# Autodesk Inventor assembly: Assembled box
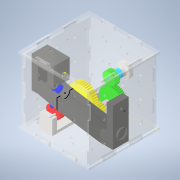
[picture p0: Inventor's stored thumbnail of the model, 180x180]
Saved by Autodesk Inventor 2021 (Build 250183000, 183)
## iProperties
Created: 2020-02-27
Part Number: Assembled box
Document SubType Name: Assembly
Designer: jstr255
Author: jstr255
## Documents named in this file (23)
- C:\Users\Jawal\Documents\UNI\PART III\Semester 1\MECHENG 334\Project A\CAD Files\Assemblies\Main 2\SPOILER_Assembly_Folder\Assembly Folder\Assembled_box.iam
- C:\Users\Jawal\Documents\UNI\PART III\Semester 1\MECHENG 334\Project A\CAD Files\Assemblies\Main 2\SPOILER_Assembly_Folder\Assembly Folder\Box_base.ipt
- C:\Users\Jawal\Documents\UNI\PART III\Semester 1\MECHENG 334\Project A\CAD Files\Assemblies\Main 2\SPOILER_Assembly_Folder\Assembly Folder\Box_side_1.ipt
- C:\Users\Jawal\Documents\UNI\PART III\Semester 1\MECHENG 334\Project A\CAD Files\Assemblies\Main 2\SPOILER_Assembly_Folder\Assembly Folder\Box_side_2.ipt
- C:\Users\Jawal\Documents\UNI\PART III\Semester 1\MECHENG 334\Project A\CAD Files\Assemblies\Main 2\SPOILER_Assembly_Folder\Assembly Folder\Box_side_3.ipt
- C:\Users\Jawal\Documents\UNI\PART III\Semester 1\MECHENG 334\Project A\CAD Files\Assemblies\Main 2\SPOILER_Assembly_Folder\Assembly Folder\Box_side_4.ipt
- C:\Users\Jawal\Documents\UNI\PART III\Semester 1\MECHENG 334\Project A\CAD Files\Assemblies\Main 2\SPOILER_Assembly_Folder\Assembly Folder\Box_top.ipt
- C:\Users\Jawal\Documents\UNI\PART III\Semester 1\MECHENG 334\Project A\CAD Files\Assemblies\Main 2\SPOILER_Assembly_Folder\Assembly Folder\Driveshaft_coupling_end.ipt
- C:\Users\Jawal\Documents\UNI\PART III\Semester 1\MECHENG 334\Project A\CAD Files\Assemblies\Main 2\SPOILER_Assembly_Folder\Assembly Folder\Input Connection.ipt
- C:\Users\Jawal\Documents\UNI\PART III\Semester 1\MECHENG 334\Project A\CAD Files\Assemblies\Main 2\SPOILER_Assembly_Folder\Assembly Folder\Block.ipt
- C:\Users\Jawal\Documents\UNI\PART III\Semester 1\MECHENG 334\Project A\CAD Files\Assemblies\Main 2\SPOILER_Assembly_Folder\Assembly Folder\bottom_part.ipt
- C:\Users\Jawal\Documents\UNI\PART III\Semester 1\MECHENG 334\Project A\CAD Files\Assemblies\Main 2\SPOILER_Assembly_Folder\Assembly Folder\entry_ramp.ipt
- C:\Users\Jawal\Documents\UNI\PART III\Semester 1\MECHENG 334\Project A\CAD Files\Assemblies\Main 2\SPOILER_Assembly_Folder\Assembly Folder\Spur Gear11.ipt
- C:\Users\Jawal\Documents\UNI\PART III\Semester 1\MECHENG 334\Project A\CAD Files\Assemblies\Main 2\SPOILER_Assembly_Folder\Assembly Folder\Spur Gear21.ipt
- C:\Users\Jawal\Documents\UNI\PART III\Semester 1\MECHENG 334\Project A\CAD Files\Assemblies\Main 2\SPOILER_Assembly_Folder\Assembly Folder\Spur Gear15.ipt
- C:\Users\Jawal\Documents\UNI\PART III\Semester 1\MECHENG 334\Project A\CAD Files\Assemblies\Main 2\SPOILER_Assembly_Folder\Assembly Folder\Spur Gear25.ipt
- C:\Users\Jawal\Documents\UNI\PART III\Semester 1\MECHENG 334\Project A\CAD Files\Assemblies\Main 2\SPOILER_Assembly_Folder\Assembly Folder\OVAAAAAL cam.ipt
- C:\Users\Jawal\Documents\UNI\PART III\Semester 1\MECHENG 334\Project A\CAD Files\Assemblies\Main 2\SPOILER_Assembly_Folder\Assembly Folder\Shaft_1.ipt
- C:\Users\Jawal\Documents\UNI\PART III\Semester 1\MECHENG 334\Project A\CAD Files\Assemblies\Main 2\SPOILER_Assembly_Folder\Assembly Folder\Shaft_2.ipt
- C:\Users\Jawal\Documents\UNI\PART III\Semester 1\MECHENG 334\Project A\CAD Files\Assemblies\Main 2\SPOILER_Assembly_Folder\Assembly Folder\Support_2A.ipt
- C:\Users\Jawal\Documents\UNI\PART III\Semester 1\MECHENG 334\Project A\CAD Files\Assemblies\Main 2\SPOILER_Assembly_Folder\Assembly Folder\Support_2B.ipt
- C:\Users\Jawal\Documents\UNI\PART III\Semester 1\MECHENG 334\Project A\CAD Files\Assemblies\Main 2\SPOILER_Assembly_Folder\Assembly Folder\Support_1B.ipt
- C:\Users\Jawal\Documents\UNI\PART III\Semester 1\MECHENG 334\Project A\CAD Files\Assemblies\Main 2\SPOILER_Assembly_Folder\Assembly Folder\Support_1A.ipt
## Components (22 placed, 20 different names)
1. Box_base:1 — Mate:1, Mate:2, Mate:3, Mate:4, Mate:5, Mate:6, Mate:7, Mate:8, Mate:9, Mate:10, Flush:4, Mate:43, Cylindrical:1, Rigid:29, Rigid:31
2. Box_side_1:1 — Mate:1, Mate:2, Mate:3, Flush:1, Mate:14, Rotational:1, Rigid:33
3. Box_side_2:1 — Mate:4, Mate:5, Mate:6, Mate:13, Rigid:17
4. Box_side_3:1 — Mate:7, Mate:8, Mate:9, Mate:11
5. Box_side_4:1 — Mate:10, Mate:11, Flush:1, Mate:12, Flush:2, Flush:14, Flush:15, Flush:18, Rigid:23, Mate:40, Mate:42
6. Box_top:1 — Mate:12, Mate:13, Mate:14
7. Driveshaft_coupling_end:2 — Rotational:1, Mate:15, Mate:16, Mate:17, Angle:1
8. Input Connection:1 — Mate:15, Mate:16, Mate:17, Rigid:24
9. Block:1 — Mate:44, Mate:45, Transitional:1
10. bottom_part:1 — Rigid:17
11. entry_ramp:1 — Rigid:23, Mate:44, Mate:45
12. Spur Gear1:1 — Flush:19, Mate:39, Mate:40, Rotation:1, Mate:46, Rigid:34
13. Spur Gear2:3 — Rigid:24, Flush:19, Mate:39, Rotation:1
14. Spur Gear1:2 — Flush:20, Rotation:2, Mate:42, Mate:43, Rigid:27
15. Spur Gear2:5 — Flush:20, Rotation:2, Mate:46, Rigid:35
16. OVAAAAAL cam:1 — Rigid:30, Transitional:1
17. Shaft_1:1 — Rigid:34, Rigid:35
18. Support_2A:1 — Cylindrical:1
19. Shaft_2:1 — Rigid:27, Rigid:30
20. Support_2B:1 — Rigid:29
21. Support_1B:1 — Rigid:31
22. Support_1A:1 — Rigid:33
## Relationships (48: Mate 24, WeldJoint 10, Flush 8, RelateRotation 2, RevoluteJoint 1, Angle 1, CylindricalJoint 1, Transitional 1)
- Mate:1: Box_base:1 ↔ Box_side_1:1
- Mate:2: Box_base:1 ↔ Box_side_1:1
- Mate:3: Box_base:1 ↔ Box_side_1:1
- Mate:4: Box_base:1 ↔ Box_side_2:1
- Mate:5: Box_base:1 ↔ Box_side_2:1
- Mate:6: Box_base:1 ↔ Box_side_2:1
- Mate:7: Box_base:1 ↔ Box_side_3:1
- Mate:8: Box_base:1 ↔ Box_side_3:1
- Mate:9: Box_base:1 ↔ Box_side_3:1
- Mate:10: Box_base:1 ↔ Box_side_4:1
- Mate:11: Box_side_3:1 ↔ Box_side_4:1
- Flush:1: Box_side_1:1 ↔ Box_side_4:1
- Mate:12: Box_side_4:1 ↔ Box_top:1
- Mate:13: Box_side_2:1 ↔ Box_top:1
- Mate:14: Box_side_1:1 ↔ Box_top:1
- Rotational:1 [RevoluteJoint]: Box_side_1:1 ↔ Driveshaft_coupling_end:2
- Mate:15: Driveshaft_coupling_end:2 ↔ Input Connection:1
- Mate:16: Driveshaft_coupling_end:2 ↔ Input Connection:1
- Mate:17: Driveshaft_coupling_end:2 ↔ Input Connection:1
- Flush:2 (50 mm): Box_side_4:1
- Flush:4 (50 mm): Box_base:1
- Flush:14 (27.503 mm): Box_side_4:1
- Angle:1 (0 deg): Driveshaft_coupling_end:2
- Flush:15 (27.503 mm): Box_side_4:1
- Flush:18 (27.503 mm): Box_side_4:1
- Rigid:17 [WeldJoint]: Box_side_2:1 ↔ bottom_part:1
- Rigid:23 [WeldJoint]: Box_side_4:1 ↔ entry_ramp:1
- Rigid:24 [WeldJoint]: Input Connection:1 ↔ Spur Gear2:3
- Flush:19: Spur Gear1:1 ↔ Spur Gear2:3
- Mate:39 (28.8 mm): Spur Gear1:1 ↔ Spur Gear2:3
- Mate:40 (53.983 mm): Box_side_4:1 ↔ Spur Gear1:1
- Flush:20: Spur Gear1:2 ↔ Spur Gear2:5
- Rotation:1 [RelateRotation] (0.5 ul): Spur Gear1:1 ↔ Spur Gear2:3
- Rotation:2 [RelateRotation] (4 ul): Spur Gear1:2 ↔ Spur Gear2:5
- Mate:42 (28.613 mm): Box_side_4:1 ↔ Spur Gear1:2
- Mate:43 (22.877 mm): Box_base:1 ↔ Spur Gear1:2
- Mate:44 (0.5 mm): Block:1 ↔ entry_ramp:1
- Mate:45 (0.5 mm): Block:1 ↔ entry_ramp:1
- Cylindrical:1: Box_base:1 ↔ Support_2A:1
- Rigid:27 [WeldJoint] (16 mm): Spur Gear1:2 ↔ Shaft_2:1
- Rigid:29 [WeldJoint]: Box_base:1 ↔ Support_2B:1
- Rigid:30 [WeldJoint] (-9.5 mm): OVAAAAAL cam:1 ↔ Shaft_2:1
- Transitional:1: Block:1 ↔ OVAAAAAL cam:1
- Rigid:31 [WeldJoint]: Box_base:1 ↔ Support_1B:1
- Mate:46 (14 mm): Spur Gear1:1 ↔ Spur Gear2:5
- Rigid:33 [WeldJoint]: Box_side_1:1 ↔ Support_1A:1
- Rigid:34 [WeldJoint] (6 mm): Spur Gear1:1 ↔ Shaft_1:1
- Rigid:35 [WeldJoint] (6.5 mm): Spur Gear2:5 ↔ Shaft_1:1
